# Autodesk Inventor assembly: ECoG_holder_4p0
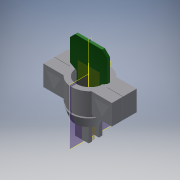
[picture p0: Inventor's stored thumbnail of the model, 180x180]
Saved by Autodesk Inventor 2017 (Build 210142000, 142)
## iProperties
Created: 2016-11-02
Part Number: ECoG_holder_4p0
Document SubType Name: Assembly
Designer: Camilo
Author: Camilo
## Documents named in this file (3)
- Z:\Github\AgingTests\3D parts\ECoG holder_4p0\ECoG_holder_4p0.iam
- Z:\Dropbox\Maharbiz Lab\Projects\SiC ECoG\Aging tests\3D parts\ECoG holder_3p\32ch_ECoG_assembled_3p0.iam
- Z:\Github\AgingTests\3D parts\ECoG holder_4p0\ECoG_holder_4p0.ipt
## Components (2 placed, 2 different names)
1. 32ch_ECoG_assembled_3p0:1 [sub-assembly] — Mate:1, Mate:2, Flush:1, Flush:2
2. ECoG_holder_4p0:1 — Flush:2
## Relationships (4: Mate 2, Flush 2)
- Mate:1: 32ch_ECoG_assembled_3p0:1
- Mate:2: 32ch_ECoG_assembled_3p0:1
- Flush:1: 32ch_ECoG_assembled_3p0:1
- Flush:2: 32ch_ECoG_assembled_3p0:1 ↔ ECoG_holder_4p0:1
